# Autodesk Inventor assembly: 肩_1
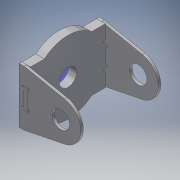
[picture p0: Inventor's stored thumbnail of the model, 180x180]
Saved by Autodesk Inventor 2018 (Build 220112000, 112)
## iProperties
Created: 2016-05-05
Part Number: 肩_1
Document SubType Name: Assembly
Designer: hiroaki
Mass: 31.2319 g
Surface Area: 187.261 cm^2
Volume: 14.2636 cm^3
Density: 2.18962 g/cm^3
Author: hiroaki
## Documents named in this file (3)
- Z:\OPR\OpenPlatform_ver1_0\上半身\腕\肩_1.iam
- Z:\OPR\OpenPlatform_ver1_0\上半身\腕\肩_メインフレーム_1_1.ipt
- Z:\OPR\OpenPlatform_ver1_0\上半身\腕\肩_サブフレーム_1_1.ipt
## Components (3 placed, 2 different names)
1. 肩_メインフレーム_1_1:1 — 挿入:1, 挿入:2, 挿入:3, 挿入:4
2. 肩_サブフレーム_1_1:1 — 挿入:3, 挿入:4
3. 肩_サブフレーム_1_1:2 — 挿入:1, 挿入:2
## Relationships (4: Insert 4)
- 挿入:1 [Insert]: 肩_メインフレーム_1_1:1 ↔ 肩_サブフレーム_1_1:2
- 挿入:2 [Insert]: 肩_メインフレーム_1_1:1 ↔ 肩_サブフレーム_1_1:2
- 挿入:3 [Insert]: 肩_メインフレーム_1_1:1 ↔ 肩_サブフレーム_1_1:1
- 挿入:4 [Insert]: 肩_メインフレーム_1_1:1 ↔ 肩_サブフレーム_1_1:1
